# Autodesk Inventor assembly: 2 in Top Block WCP-0418
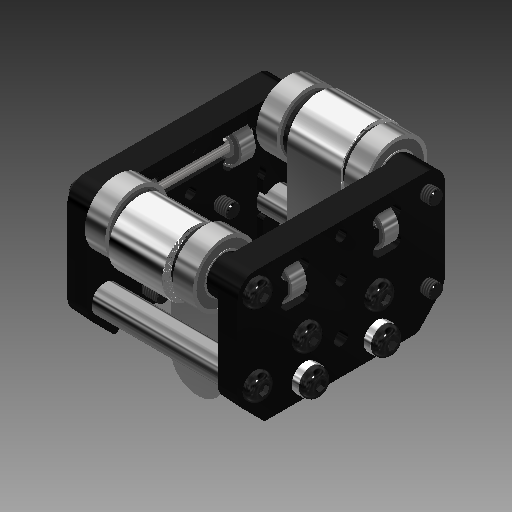
[picture p0: Inventor's stored thumbnail of the model, 512x512]
Saved by Autodesk Inventor 2023 (Build 270158000, 158)
## iProperties
Created: 2022-01-15
Part Number: 2 in Top Block WCP-0418
Document SubType Name: Assembly
Mass: 368.528 g
Surface Area: 613.658 cm^2
Volume: 78.706 cm^3
Density: 4.68233 g/cm^3
Revision Number: ANY
## Documents named in this file (16)
- E:\Collaborative Robots\Collaborative Part Library\Elevators\GreyT Telescope\2 in Top Block WCP-0419.iam
- E:\Collaborative Robots\Collaborative Part Library\Elevators\GreyT Telescope\Mid-small Stage\WCP-0419-004 Rev1.ipt
- E:\Collaborative Robots\Collaborative Part Library\Hardware\Spacers\Spacers & Standoffs\Aluminum Unthreaded Spacer (No. 10 x 0.094Lg x 0.375OD).ipt
- C:\Users\Cal\Desktop\Robotics\Design\Collaborative\Collaborative Parts Library\Hardware\Spacers\Spacers & Standoffs.ipt
- E:\Collaborative Robots\Collaborative Part Library\Hardware\Fasteners\Machine Screws\10-32 UNFx0.5 Button Head Cap Screw.ipt
- C:\Users\Cal\Desktop\Robotics\Design\Collaborative\Collaborative Parts Library\Hardware\Fasteners\Machine Screws.ipt
- E:\Collaborative Robots\Collaborative Part Library\Hardware\Fasteners\Machine Screws\10-32 UNFx0.375 Button Head Cap Screw.ipt
- E:\Collaborative Robots\Collaborative Part Library\Hardware\Fasteners\Machine Screws\10-32 UNFx2.5 Button Head Cap Screw.ipt
- E:\Collaborative Robots\Collaborative Part Library\Hardware\Dowel Pins\Dowel Pins\0.1875in  x 1.75in Stainless Steel Dowel Pin.ipt
- C:\Users\Cal\Desktop\Robotics\Design\Collaborative\Collaborative Parts Library\Hardware\Dowel Pins\Dowel Pins.ipt
- E:\Collaborative Robots\Collaborative Part Library\Power Transfer\Bearings and Bushings\Bearings\R3ZZ.ipt
- C:\Users\Cal\Desktop\Robotics\Design\Collaborative\Collaborative Parts Library\Power Transfer\Bearings and Bushings\Bearings.ipt
- E:\Collaborative Robots\Collaborative Part Library\Elevators\GreyT Telescope\Mid-small Stage\WCP-0419-006 Rev1.ipt
- E:\Collaborative Robots\Collaborative Part Library\Power Transfer\Bearings and Bushings\Bearings\R6.ipt
- E:\Collaborative Robots\Collaborative Part Library\Hardware\Spacers\Spacers & Standoffs\WCP Aluminum Standoff (No. 10 x 2Lg x 0.375OD).ipt
- E:\Collaborative Robots\Collaborative Part Library\Elevators\GreyT Telescope\GreyT Constant Force Spring.ipt
## Components (38 placed, 12 different names)
1. WCP-0419-004 Rev1_978 — Insert:1, Insert:2, Insert:9, Insert:10, Insert:13, Insert:14, Tangent:1, Tangent:3, Insert:23, Insert:24, Angle:1, Insert:27, Insert:29
2. WCP-0419-004 Rev1_979 — Insert:3, Insert:4, Insert:11, Insert:12, Insert:15, Insert:16, Tangent:2, Tangent:4, Insert:25, Angle:1, Insert:26, Insert:28, Insert:30, Insert:31
3. 10-32 UNFx2.5 Button Head Cap Screw:10 — Insert:13
4. 10-32 UNFx2.5 Button Head Cap Screw:11 — Insert:14
5. 10-32 UNFx2.5 Button Head Cap Screw:12 — Insert:16
6. 10-32 UNFx2.5 Button Head Cap Screw:13 — Insert:15
7. 10-32 UNFx0.375 Button Head Cap Screw:6 — Insert:9
8. 10-32 UNFx0.375 Button Head Cap Screw:7 — Insert:10
9. 10-32 UNFx0.5 Button Head Cap Screw:1 — Insert:6
10. 10-32 UNFx0.5 Button Head Cap Screw:2 — Insert:5
11. 10-32 UNFx0.5 Button Head Cap Screw:3 — Insert:7
12. 10-32 UNFx0.5 Button Head Cap Screw:4 — Insert:8
13. 10-32 UNFx0.375 Button Head Cap Screw:8 — Insert:11
14. 10-32 UNFx0.375 Button Head Cap Screw:9 — Insert:12
15. WCP-0419-006 Rev1:5 — Insert:19, Tangent:7
16. Aluminum Unthreaded Spacer (No. 10 x 0.094Lg x 0.375OD):1 — Insert:1, Insert:5
17. Aluminum Unthreaded Spacer (No. 10 x 0.094Lg x 0.375OD):2 — Insert:2, Insert:6
18. Aluminum Unthreaded Spacer (No. 10 x 0.094Lg x 0.375OD):3 — Insert:4, Insert:8
19. Aluminum Unthreaded Spacer (No. 10 x 0.094Lg x 0.375OD):4 — Insert:3, Insert:7
20. 0.1875in  x 1.75in Stainless Steel Dowel Pin:1 — Mate:1, Tangent:1, Tangent:3, Flush:2
21. R3ZZ:1 — Insert:17, Symmetry:1, Flush:1
22. R3ZZ:2 — Insert:17, Mate:1, Symmetry:1
23. 0.1875in  x 1.75in Stainless Steel Dowel Pin:2 — Tangent:2, Tangent:4
24. R3ZZ:3 — Flush:1
25. R3ZZ:4
26. R6:5 — Insert:19, Insert:26
27. WCP-0419-006 Rev1:6
28. R6:6 — Insert:27
29. WCP-0419-006 Rev1:7 — Symmetry:3, Tangent:6
30. R6:7 — Insert:29
31. WCP-0419-006 Rev1:8 — Symmetry:3
32. R6:8 — Insert:28
33. WCP Aluminum Standoff (No. 10 x 2Lg x 0.375OD):5 — Insert:23, Insert:25
34. WCP Aluminum Standoff (No. 10 x 2Lg x 0.375OD):6 — Insert:24
35. WCP Aluminum Standoff (No. 10 x 2Lg x 0.375OD):7 — Insert:30
36. WCP Aluminum Standoff (No. 10 x 2Lg x 0.375OD):8 — Insert:31
37. GreyT Constant Force Spring:1 — Tangent:6, Mate:3, Flush:3, Symmetry:4, Mate:4
38. GreyT Constant Force Spring:2 — Mate:3, Flush:3, Symmetry:4, Mate:4, Tangent:7
## Relationships (49: Insert 31, Tangent 6, Mate 4, Symmetry 4, Flush 3, Angle 1)
- Insert:1: WCP-0419-004 Rev1_978 ↔ Aluminum Unthreaded Spacer (No. 10 x 0.094Lg x 0.375OD):1
- Insert:2: WCP-0419-004 Rev1_978 ↔ Aluminum Unthreaded Spacer (No. 10 x 0.094Lg x 0.375OD):2
- Insert:3: WCP-0419-004 Rev1_979 ↔ Aluminum Unthreaded Spacer (No. 10 x 0.094Lg x 0.375OD):4
- Insert:4: WCP-0419-004 Rev1_979 ↔ Aluminum Unthreaded Spacer (No. 10 x 0.094Lg x 0.375OD):3
- Insert:5: 10-32 UNFx0.5 Button Head Cap Screw:2 ↔ Aluminum Unthreaded Spacer (No. 10 x 0.094Lg x 0.375OD):1
- Insert:6: 10-32 UNFx0.5 Button Head Cap Screw:1 ↔ Aluminum Unthreaded Spacer (No. 10 x 0.094Lg x 0.375OD):2
- Insert:7: 10-32 UNFx0.5 Button Head Cap Screw:3 ↔ Aluminum Unthreaded Spacer (No. 10 x 0.094Lg x 0.375OD):4
- Insert:8: 10-32 UNFx0.5 Button Head Cap Screw:4 ↔ Aluminum Unthreaded Spacer (No. 10 x 0.094Lg x 0.375OD):3
- Insert:9: WCP-0419-004 Rev1_978 ↔ 10-32 UNFx0.375 Button Head Cap Screw:6
- Insert:10: WCP-0419-004 Rev1_978 ↔ 10-32 UNFx0.375 Button Head Cap Screw:7
- Insert:11: WCP-0419-004 Rev1_979 ↔ 10-32 UNFx0.375 Button Head Cap Screw:8
- Insert:12: WCP-0419-004 Rev1_979 ↔ 10-32 UNFx0.375 Button Head Cap Screw:9
- Insert:13: WCP-0419-004 Rev1_978 ↔ 10-32 UNFx2.5 Button Head Cap Screw:10
- Insert:14: WCP-0419-004 Rev1_978 ↔ 10-32 UNFx2.5 Button Head Cap Screw:11
- Insert:15: WCP-0419-004 Rev1_979 ↔ 10-32 UNFx2.5 Button Head Cap Screw:13
- Insert:16: WCP-0419-004 Rev1_979 ↔ 10-32 UNFx2.5 Button Head Cap Screw:12
- Insert:17 (27.6352 mm): R3ZZ:1 ↔ R3ZZ:2
- Mate:1: 0.1875in  x 1.75in Stainless Steel Dowel Pin:1 ↔ R3ZZ:2
- Symmetry:1: R3ZZ:1 ↔ R3ZZ:2
- [Insert] (27.6352 mm): R3ZZ:3 ↔ R3ZZ:4
- [Mate]: 0.1875in  x 1.75in Stainless Steel Dowel Pin:2 ↔ R3ZZ:4
- [Symmetry]: R3ZZ:3 ↔ R3ZZ:4
- Flush:1: R3ZZ:1 ↔ R3ZZ:3
- Tangent:1: WCP-0419-004 Rev1_978 ↔ 0.1875in  x 1.75in Stainless Steel Dowel Pin:1
- Tangent:2: WCP-0419-004 Rev1_979 ↔ 0.1875in  x 1.75in Stainless Steel Dowel Pin:2
- Tangent:3: WCP-0419-004 Rev1_978 ↔ 0.1875in  x 1.75in Stainless Steel Dowel Pin:1
- Tangent:4: WCP-0419-004 Rev1_979 ↔ 0.1875in  x 1.75in Stainless Steel Dowel Pin:2
- Flush:2: 0.1875in  x 1.75in Stainless Steel Dowel Pin:1
- Insert:19: WCP-0419-006 Rev1:5 ↔ R6:5
- [Insert]: WCP-0419-006 Rev1:6 ↔ R6:6
- [Insert]: WCP-0419-006 Rev1:7 ↔ R6:7
- [Insert]: WCP-0419-006 Rev1:8 ↔ R6:8
- Insert:23: WCP-0419-004 Rev1_978 ↔ WCP Aluminum Standoff (No. 10 x 2Lg x 0.375OD):5
- Insert:24: WCP-0419-004 Rev1_978 ↔ WCP Aluminum Standoff (No. 10 x 2Lg x 0.375OD):6
- Insert:25: WCP-0419-004 Rev1_979 ↔ WCP Aluminum Standoff (No. 10 x 2Lg x 0.375OD):5
- Angle:1 (0 deg): WCP-0419-004 Rev1_978 ↔ WCP-0419-004 Rev1_979
- Insert:26: WCP-0419-004 Rev1_979 ↔ R6:5
- Insert:27: WCP-0419-004 Rev1_978 ↔ R6:6
- Insert:28: WCP-0419-004 Rev1_979 ↔ R6:8
- Insert:29: WCP-0419-004 Rev1_978 ↔ R6:7
- Insert:30: WCP-0419-004 Rev1_979 ↔ WCP Aluminum Standoff (No. 10 x 2Lg x 0.375OD):7
- Insert:31: WCP-0419-004 Rev1_979 ↔ WCP Aluminum Standoff (No. 10 x 2Lg x 0.375OD):8
- Symmetry:3: WCP-0419-006 Rev1:7 ↔ WCP-0419-006 Rev1:8
- Tangent:6: WCP-0419-006 Rev1:7 ↔ GreyT Constant Force Spring:1
- Mate:3: GreyT Constant Force Spring:1 ↔ GreyT Constant Force Spring:2
- Flush:3: GreyT Constant Force Spring:1 ↔ GreyT Constant Force Spring:2
- Symmetry:4: GreyT Constant Force Spring:1 ↔ GreyT Constant Force Spring:2
- Mate:4 (38.1 mm): GreyT Constant Force Spring:1 ↔ GreyT Constant Force Spring:2
- Tangent:7: WCP-0419-006 Rev1:5 ↔ GreyT Constant Force Spring:2
## Named parameters: d18_d16 = 27.6352 mm, d19_d17 = 0 mm, d27_d26 = 0 mm, d28_d26 = 0 mm, d29_d26 = 0 mm
